# Autodesk Inventor assembly: SpeakerAssembled
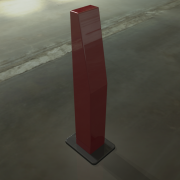
[picture p0: Inventor's stored thumbnail of the model, 180x180]
Saved by Autodesk Inventor 2015 (Build 190159000, 159)
## iProperties
Created: 2015-02-02
Part Number: SpeakerAssembled
Document SubType Name: Assembly
Designer: rubidium
Author: rubidium
## Documents named in this file (10)
- L:\Git\ModAudio\SpeakerAssembled.iam
- L:\Git\ModAudio\la_side.ipt
- L:\Git\ModAudio\topbottomsquare.ipt
- L:\Git\ModAudio\speakerfront.ipt
- L:\Git\ModAudio\toprectangle.ipt
- L:\Git\ModAudio\lowerback.ipt
- L:\Git\ModAudio\topback.ipt
- L:\Git\ModAudio\speaker_6_5in.ipt
- L:\Git\ModAudio\tweets.ipt
- L:\Git\ModAudio\base.ipt
## Components (35 placed, 9 different names)
1. base:1 — Mate:12, Flush:13, Flush:14, Flush:15, Flush:16, Flush:17
2. la_side:1 — Flush:1, Flush:2, Mate:1, Flush:4, Flush:6, Flush:7, Flush:9, Flush:10, Flush:11, Mate:9, Flush:12
3. la_side:2 — Flush:1, Flush:2, Mate:2, Flush:3, Mate:4, Mate:8, Mate:10, Flush:13
4. topbottomsquare:1 — Mate:1, Mate:2, Flush:3, Mate:5, Flush:5, Flush:6, Flush:7, Mate:12
5. speakerfront:1 — Mate:4, Mate:5, Flush:4, Flush:5, Mate:11, Insert:1, Insert:2, Insert:3, Insert:4, Insert:5, Insert:6, Insert:7, Insert:8, Insert:9, Insert:10, Insert:11, Insert:12, Insert:13, Insert:14, Insert:15, Insert:16, Insert:17, Insert:18, Insert:19, Insert:20, Insert:21, Insert:22, Insert:23, Insert:24, Insert:25, Insert:26, Insert:27
6. toprectangle:1 — Flush:12, Mate:10, Mate:11
7. lowerback:1 — Flush:9, Flush:10, Mate:8, Flush:14
8. topback:1 — Flush:11, Mate:9
9. speaker_6_5in:1 — Insert:1
10. speaker_6_5in:2 — Insert:2
11. speaker_6_5in:3 — Insert:3
12. speaker_6_5in:4 — Insert:4
13. speaker_6_5in:5 — Insert:5
14. speaker_6_5in:6 — Insert:6
15. speaker_6_5in:7 — Insert:7
16. speaker_6_5in:8 — Insert:8
17. speaker_6_5in:9 — Insert:9
18. tweets:1 — Insert:11
19. tweets:2 — Insert:10
20. tweets:3 — Insert:12
21. tweets:4 — Insert:13
22. tweets:5 — Insert:14
23. tweets:6 — Insert:15
24. tweets:7 — Insert:16
25. tweets:8 — Insert:17
26. tweets:9 — Insert:18
27. tweets:10 — Insert:19
28. tweets:11 — Insert:20
29. tweets:12 — Insert:21
30. tweets:13 — Insert:22
31. tweets:14 — Insert:23
32. tweets:15 — Insert:24
33. tweets:17 — Insert:25
34. tweets:18 — Insert:26
35. tweets:19 — Insert:27
## Relationships (52: Insert 27, Flush 16, Mate 9)
- Flush:1: la_side:1 ↔ la_side:2
- Flush:2: la_side:1 ↔ la_side:2
- Mate:1: la_side:1 ↔ topbottomsquare:1
- Mate:2: la_side:2 ↔ topbottomsquare:1
- Flush:3: la_side:2 ↔ topbottomsquare:1
- Mate:4: la_side:2 ↔ speakerfront:1
- Mate:5: topbottomsquare:1 ↔ speakerfront:1
- Flush:4: la_side:1 ↔ speakerfront:1
- Flush:5: topbottomsquare:1 ↔ speakerfront:1
- Flush:6: la_side:1 ↔ topbottomsquare:1
- Flush:7: la_side:1 ↔ topbottomsquare:1
- Flush:9: la_side:1 ↔ lowerback:1
- Flush:10: la_side:1 ↔ lowerback:1
- Mate:8: la_side:2 ↔ lowerback:1
- Flush:11: la_side:1 ↔ topback:1
- Mate:9: la_side:1 ↔ topback:1
- Flush:12: la_side:1 ↔ toprectangle:1
- Mate:10: la_side:2 ↔ toprectangle:1
- Mate:11: speakerfront:1 ↔ toprectangle:1
- Insert:1: speakerfront:1 ↔ speaker_6_5in:1
- Insert:2: speakerfront:1 ↔ speaker_6_5in:2
- Insert:3: speakerfront:1 ↔ speaker_6_5in:3
- Insert:4: speakerfront:1 ↔ speaker_6_5in:4
- Insert:5: speakerfront:1 ↔ speaker_6_5in:5
- Insert:6: speakerfront:1 ↔ speaker_6_5in:6
- Insert:7: speakerfront:1 ↔ speaker_6_5in:7
- Insert:8: speakerfront:1 ↔ speaker_6_5in:8
- Insert:9: speakerfront:1 ↔ speaker_6_5in:9
- Insert:10: speakerfront:1 ↔ tweets:2
- Insert:11: speakerfront:1 ↔ tweets:1
- Insert:12: speakerfront:1 ↔ tweets:3
- Insert:13: speakerfront:1 ↔ tweets:4
- Insert:14: speakerfront:1 ↔ tweets:5
- Insert:15: speakerfront:1 ↔ tweets:6
- Insert:16: speakerfront:1 ↔ tweets:7
- Insert:17: speakerfront:1 ↔ tweets:8
- Insert:18: speakerfront:1 ↔ tweets:9
- Insert:19: speakerfront:1 ↔ tweets:10
- Insert:20: speakerfront:1 ↔ tweets:11
- Insert:21: speakerfront:1 ↔ tweets:12
- Insert:22: speakerfront:1 ↔ tweets:13
- Insert:23: speakerfront:1 ↔ tweets:14
- Insert:24: speakerfront:1 ↔ tweets:15
- Insert:25: speakerfront:1 ↔ tweets:17
- Insert:26: speakerfront:1 ↔ tweets:18
- Insert:27: speakerfront:1 ↔ tweets:19
- Mate:12: base:1 ↔ topbottomsquare:1
- Flush:13 (82.55 mm): base:1 ↔ la_side:2
- Flush:14 (152.4 mm): base:1 ↔ lowerback:1
- Flush:15: base:1
- Flush:16: base:1
- Flush:17: base:1
